# Autodesk Inventor assembly: FullFrame.003
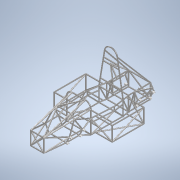
[picture p0: Inventor's stored thumbnail of the model, 180x180]
Saved by Autodesk Inventor 2021 (Build 250183000, 183)
## iProperties
Created: 2020-11-18
Part Number: FullFrame.003
Document SubType Name: Assembly
Designer: qv17m
_SolveAssemblyDoc: Frame Generator Solve Assembly
_Version: 25.0.0
Author: qv17m
## Documents named in this file (4)
- C:\Users\qv17m\Documents\Inventor\FSAE\LafayetteCollegeRearFrame.003\FullFrame.003.iam
- C:\Users\qv17m\Documents\Inventor\FSAE\LafayetteCollegeRearFrame.003\RearFrame.003.ipt
- C:\Users\qv17m\Documents\Inventor\FSAE\LafayetteCollegeRearFrame.003\FrontFrame.003.ipt
- C:\Users\qv17m\Documents\Inventor\FSAE\LafayetteCollegeRearFrame.003\FullFrame.003\Frame\Frame 1605682370645.iam
## Components (3 placed, 3 different names)
1. RearFrame.003:1 — Mate:1
2. FrontFrame.003:1 — Mate:1
3. Frame 1605682370645:1 [sub-assembly]
## Relationships (1: Mate 1)
- Mate:1: RearFrame.003:1 ↔ FrontFrame.003:1
